# Autodesk Inventor assembly: Medium Conveyor-Belt Link
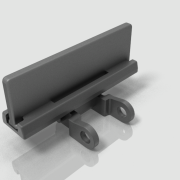
[picture p0: Inventor's stored thumbnail of the model, 180x180]
Saved by Autodesk Inventor 2013 (Build 170138000, 138)
## iProperties
Category: Motion
Company: Super Sonic Sparks, Team 24
Vendor: VEX Robotics, Inc.
Document SubType Name: Assembly
Designer: Jordan Kiesel
Catalog Web Link: vexrobotics.com/276-2214.html
Description: For use in constructing conveyor belt type mechanisms.
Author: Jordan Kiesel
Title: Medium Conveyor-Belt Link
Comments: For use in constructing conveyor belt type mechanisms. ▷ Compatible with Tank Tread Kit, High Strength Chain & Sprockets.
## Documents named in this file (3)
- C:\Users\WEBCAST2\Documents\New VEX CAD Parts\Chain & Tank Tread\Short Conveyor-Belt Link.iam
- C:\Users\WEBCAST2\Documents\New VEX CAD Parts\Chain & Tank Tread\Assembly Parts\Conveyor-Belt Links\Conveyor-Belt Base Link.ipt
- C:\Users\WEBCAST2\Documents\New VEX CAD Parts\Chain & Tank Tread\Assembly Parts\Conveyor-Belt Links\Short Conveyor-Belt Insert.ipt
## Components (2 placed, 2 different names)
1. Conveyor-Belt Base Link:1 — Mate:1, Mate:2, Flush:1
2. Short Conveyor-Belt Insert:1 — Mate:1, Mate:2, Flush:1
## Relationships (3: Mate 2, Flush 1)
- Mate:1: Conveyor-Belt Base Link:1 ↔ Short Conveyor-Belt Insert:1
- Mate:2: Conveyor-Belt Base Link:1 ↔ Short Conveyor-Belt Insert:1
- Flush:1: Conveyor-Belt Base Link:1 ↔ Short Conveyor-Belt Insert:1
